# Autodesk Inventor assembly: lab powersupply
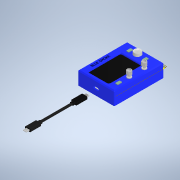
[picture p0: Inventor's stored thumbnail of the model, 180x180]
Saved by Autodesk Inventor 2022 (Build 260153000, 153)
## iProperties
Company: Open CASCADE
Created: 2021-01-26
Part Number: lab powersupply
Document SubType Name: Assembly
Designer: simen
Description: Open CASCADE Model
Authority: Unknown
Sending System: Open CASCADE 6.8
Preprocessor: Open CASCADE STEP processor 6.8
Author: Author
Title: Open CASCADE Shape Model
## Documents named in this file (16)
- C:\Users\simen\Documents\powersupply\encosure\inventor\rev1\lab powersupply.iam
- C:\Users\simen\Documents\powersupply\encosure\inventor\rev1\Frontpanel.ipt
- C:\Users\simen\Documents\powersupply\encosure\inventor\rev1\Battery.ipt
- C:\Users\simen\Documents\powersupply\encosure\inventor\rev1\Encoder knob.ipt
- C:\Users\simen\Documents\powersupply\encosure\inventor\rev1\button.ipt
- C:\Users\simen\Documents\powersupply\encosure\inventor\rev1\Display.ipt
- C:\Users\simen\Documents\powersupply\encosure\inventor\rev1\LOGO.ipt
- C:\Users\simen\Documents\powersupply\encosure\inventor\rev1\ON_Off_switch.ipt
- C:\Users\simen\Downloads\70799717.ipt
- C:\Users\simen\Downloads\111-2223-001.ipt
- C:\Users\simen\Documents\powersupply\encosure\inventor\rev1\Bottom_lid.ipt
- C:\Users\simen\Documents\M30X170C.ipt
- C:\Users\simen\Documents\powersupply\pcb\Powersupply\3d\PCB1_2.iam
- C:\Users\simen\Documents\powersupply\encosure\inventor\rev1\display_holder.ipt
- C:\Users\simen\Documents\powersupply\encosure\inventor\rev1\battery_holder.ipt
- C:\Users\simen\Downloads\encoder_knob_custom.ipt
## Components (18 placed, 15 different names)
1. Frontpanel:1 — Flush:2, Mate:16, Mate:19, Mate:23, Mate:24, Mate:29, Mate:30, Mate:35, Mate:37, Mate:39, Mate:40, Mate:43, Mate:44, Mate:45, Mate:46, Flush:3, Mate:47, Mate:48, Mate:49, Mate:50, Mate:51, Mate:62, Mate:66, Mate:67, Mate:68, Mate:69, Mate:70, Mate:71
2. Battery:1 — Flush:3
3. Encoder knob(OEJNI-50-2-7):1 — Flush:2, Mate:40
4. button:1 — Mate:35, Mate:66, Mate:67
5. button:2 — Mate:39, Mate:45, Mate:46
6. button:3 — Mate:37, Mate:43, Mate:44
7. Display:1 — Mate:16, Mate:47, Mate:48, Mate:72, Mate:73, Flush:4
8. LOGO:1
9. ON_Off_switch:1 — Mate:19, Mate:68
10. 70799717:1
11. 111-2223-001:1 — Mate:24, Mate:30
12. 111-2223-001:2 — Mate:23, Mate:29
13. Bottom_lid:1 — Mate:49, Mate:50, Mate:51
14. M30X170C:1 — Mate:62
15. PCB1_2:2 [sub-assembly] — Mate:69, Mate:70, Mate:71, Mate:74, Mate:77, Mate:78
16. display_holder:1 — Mate:72, Mate:73, Flush:4, Flush:76
17. battery_holder:1 — Mate:74, Flush:76
18. encoder_knob_custom:1 — Mate:77, Mate:78
## Relationships (35: Mate 31, Flush 4)
- Flush:2 (0.2 mm): Frontpanel:1 ↔ Encoder knob(OEJNI-50-2-7):1
- Mate:16 (0.05 mm): Frontpanel:1 ↔ Display:1
- Mate:19: Frontpanel:1 ↔ ON_Off_switch:1
- Mate:23: Frontpanel:1 ↔ 111-2223-001:2
- Mate:24: Frontpanel:1 ↔ 111-2223-001:1
- Mate:29: Frontpanel:1 ↔ 111-2223-001:2
- Mate:30: Frontpanel:1 ↔ 111-2223-001:1
- Mate:35: Frontpanel:1 ↔ button:1
- Mate:37: Frontpanel:1 ↔ button:3
- Mate:39: Frontpanel:1 ↔ button:2
- Mate:40: Frontpanel:1 ↔ Encoder knob(OEJNI-50-2-7):1
- Mate:43 (0.25 mm): Frontpanel:1 ↔ button:3
- Mate:44 (0.25 mm): Frontpanel:1 ↔ button:3
- Mate:45 (0.25 mm): Frontpanel:1 ↔ button:2
- Mate:46 (0.25 mm): Frontpanel:1 ↔ button:2
- Flush:3: Frontpanel:1 ↔ Battery:1
- Mate:47 (6.5 mm): Frontpanel:1 ↔ Display:1
- Mate:48 (1 mm): Frontpanel:1 ↔ Display:1
- Mate:49: Frontpanel:1 ↔ Bottom_lid:1
- Mate:50: Frontpanel:1 ↔ Bottom_lid:1
- Mate:51: Frontpanel:1 ↔ Bottom_lid:1
- Mate:62: Frontpanel:1 ↔ M30X170C:1
- Mate:66 (0.25 mm): Frontpanel:1 ↔ button:1
- Mate:67 (0.25 mm): Frontpanel:1 ↔ button:1
- Mate:68 (0.25 mm): Frontpanel:1 ↔ ON_Off_switch:1
- Mate:69: Frontpanel:1 ↔ PCB1_2:2
- Mate:70: Frontpanel:1 ↔ PCB1_2:2
- Mate:71: Frontpanel:1 ↔ PCB1_2:2
- Mate:72: Display:1 ↔ display_holder:1
- Mate:73: Display:1 ↔ display_holder:1
- Flush:4 (14.3 mm): Display:1 ↔ display_holder:1
- Mate:74: PCB1_2:2 ↔ battery_holder:1
- Flush:76 (13 mm): display_holder:1 ↔ battery_holder:1
- Mate:77: PCB1_2:2 ↔ encoder_knob_custom:1
- Mate:78: PCB1_2:2 ↔ encoder_knob_custom:1
